# Autodesk Inventor assembly: Assembly
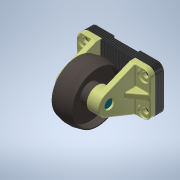
[picture p0: Inventor's stored thumbnail of the model, 180x180]
Saved by Autodesk Inventor 2020 (Build 240168000, 168)
## iProperties
Created: 2021-06-13
Part Number: Assembly
Document SubType Name: Assembly
Designer: joelm
Mass: 3792.34 g
Surface Area: 1159.89 cm^2
Volume: 474.043 cm^3
Density: 8 g/cm^3
Author: joelm
## Documents named in this file (11)
- D:\Carreer 4.1\Manufacturing Tech\DieSetProject-20210729T070551Z-001\DieSetProject\DieSet\Assembly.iam
- D:\Carreer 4.1\Manufacturing Tech\DieSetProject-20210729T070551Z-001\DieSetProject\DieSet\axle.ipt
- D:\Carreer 4.1\Manufacturing Tech\DieSetProject-20210729T070551Z-001\DieSetProject\DieSet\axleSupport.ipt
- D:\Carreer 4.1\Manufacturing Tech\DieSetProject-20210729T070551Z-001\DieSetProject\DieSet\topPlate.ipt
- D:\Carreer 4.1\Manufacturing Tech\DieSetProject-20210729T070551Z-001\DieSetProject\DieSet\wheel.ipt
- D:\Carreer 4.1\Manufacturing Tech\DieSetProject-20210729T070551Z-001\DieSetProject\DieSet\Assembly\AIP\FEA\doj74jy1s.fins
- D:\Carreer 4.1\Manufacturing Tech\DieSetProject-20210729T070551Z-001\DieSetProject\DieSet\Assembly\AIP\FEA\doj74jy1s.fsat
- D:\Carreer 4.1\Manufacturing Tech\DieSetProject-20210729T070551Z-001\DieSetProject\DieSet\Assembly\AIP\FEA\doj74jy2o.ftes
- D:\Carreer 4.1\Manufacturing Tech\DieSetProject-20210729T070551Z-001\DieSetProject\DieSet\Assembly\AIP\FEA\doj74jy2o.fwiz
- D:\Carreer 4.1\Manufacturing Tech\DieSetProject-20210729T070551Z-001\DieSetProject\DieSet\Assembly\AIP\FEA\doj74jyhs.fmsh
- D:\Carreer 4.1\Manufacturing Tech\DieSetProject-20210729T070551Z-001\DieSetProject\DieSet\Assembly\AIP\FEA\doj74jyht.fres
## Components (5 placed, 4 different names)
1. axle:1 — Mate:1, Mate:2, Flush:1
2. axleSupport:1 — Mate:2, Flush:1, Mate:4, Mate:6, Mate:7, Flush:2
3. topPlate:1 — Mate:5, Mate:6, Mate:7, Flush:2, Flush:3
4. wheel:1 — Mate:1, Mate:3, Mate:4
5. axleSupport:2 — Mate:3, Mate:5, Flush:3
## Relationships (10: Mate 7, Flush 3)
- Mate:1: axle:1 ↔ wheel:1
- Mate:2: axle:1 ↔ axleSupport:1
- Mate:3: wheel:1 ↔ axleSupport:2
- Flush:1 (-2 mm): axle:1 ↔ axleSupport:1
- Mate:4: axleSupport:1 ↔ wheel:1
- Mate:5: topPlate:1 ↔ axleSupport:2
- Mate:6: axleSupport:1 ↔ topPlate:1
- Mate:7: axleSupport:1 ↔ topPlate:1
- Flush:2: axleSupport:1 ↔ topPlate:1
- Flush:3: topPlate:1 ↔ axleSupport:2
## Named parameters: sa_0 = 981, sa_1 = 1e+07
note: some values were not read from the file. Shown as the stored number, unit unknown: "sa_0", "sa_1".
